# Autodesk Inventor assembly: objectRetrieval
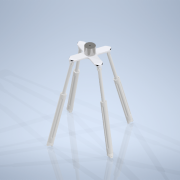
[picture p0: Inventor's stored thumbnail of the model, 180x180]
Saved by Autodesk Inventor 2022 (Build 260153000, 153)
## iProperties
Created: 2022-04-28
Part Number: objectRetrieval
Document SubType Name: Assembly
Designer: Dahway
Author: Dahway
## Documents named in this file (6)
- C:\Users\Dahway\Documents\GitHub\GMU-RobotX-Mechanical\Object Retrieval\V3\objectRetrieval.iam
- C:\Users\Dahway\Documents\GitHub\GMU-RobotX-Mechanical\Object Retrieval\V3\armLower.ipt
- C:\Users\Dahway\Documents\GitHub\GMU-RobotX-Mechanical\Object Retrieval\V3\armPlug.ipt
- C:\Users\Dahway\Documents\GitHub\GMU-RobotX-Mechanical\Object Retrieval\V3\armUpper.ipt
- C:\Users\Dahway\Documents\GitHub\GMU-RobotX-Mechanical\Object Retrieval\V3\equipPlate.ipt
- C:\Users\Dahway\Documents\GitHub\GMU-RobotX-Mechanical\Object Retrieval\Mock ups\Electromagnet.ipt
## Components (14 placed, 5 different names)
1. equipPlate:1 — Mate:7, Mate:8, Mate:9, Mate:10, Mate:11, Mate:12
2. Electromagnet:1 — Mate:11, Mate:12
3. armLower:1 — Mate:1, Mate:2, Mate:6, Mate:8, Mate:9, Mate:10
4. armPlug:1 — Mate:3, Mate:4, Mate:5
5. armUpper:1 — Mate:1, Mate:2, Mate:3, Mate:4, Mate:5, Mate:6
6. armLower:2
7. armPlug:2
8. armUpper:2
9. armLower:3
10. armPlug:3
11. armUpper:3
12. armLower:4
13. armPlug:4
14. armUpper:4
## Component patterns: (4 elements, first: armLower:1 + armPlug:1 + armUpper:1)
## Relationships (12: Mate 12)
- Mate:1: armLower:1 ↔ armUpper:1
- Mate:2: armLower:1 ↔ armUpper:1
- Mate:3: armPlug:1 ↔ armUpper:1
- Mate:4: armPlug:1 ↔ armUpper:1
- Mate:5: armPlug:1 ↔ armUpper:1
- Mate:6: armLower:1 ↔ armUpper:1
- Mate:7: equipPlate:1
- Mate:8 (0.508 mm): equipPlate:1 ↔ armLower:1
- Mate:9 (2.54 mm): equipPlate:1 ↔ armLower:1
- Mate:10: equipPlate:1 ↔ armLower:1
- Mate:11: equipPlate:1 ↔ Electromagnet:1
- Mate:12: equipPlate:1 ↔ Electromagnet:1
